# Autodesk Inventor assembly: Assembly
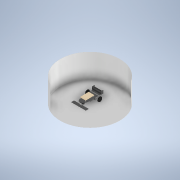
[picture p0: Inventor's stored thumbnail of the model, 180x180]
Saved by Autodesk Inventor 2022 (Build 260153000, 153)
## iProperties
Created: 2021-07-05
Part Number: Assembly
Document SubType Name: Assembly
Designer: ken
Author: ken
## Documents named in this file (12)
- G:\マイドライブ\Projects\lineTracer\inventor\LineTracer.iam
- G:\マイドライブ\Projects\lineTracer\inventor\Tamiya-doubleGearbox.ipt
- G:\マイドライブ\Projects\lineTracer\inventor\Tamiya-SlimTire-36mm.ipt
- G:\マイドライブ\Projects\lineTracer\inventor\Tamiya-ballcaster.ipt
- G:\マイドライブ\Projects\lineTracer\inventor\Akizuki-LineTraceSensor.ipt
- G:\マイドライブ\Projects\lineTracer\inventor\UniversalBoard-72×47.ipt
- G:\マイドライブ\Projects\lineTracer\inventor\spacer-3×10mm.ipt
- G:\マイドライブ\Projects\lineTracer\inventor\spacer-3×20mm.ipt
- G:\マイドライブ\Projects\lineTracer\inventor\18650batteryBox.ipt
- G:\マイドライブ\Projects\lineTracer\inventor\LineTracer-body.ipt
- G:\マイドライブ\Projects\lineTracer\inventor\Tamiya-doubleGearBoxStopper.ipt
- G:\マイドライブ\Projects\lineTracer\inventor\stage.ipt
## Components (17 placed, 11 different names)
1. LineTracer-body:1 — 挿入:22, 挿入:23, 挿入:28, 挿入:29, 挿入:30, 挿入:31, 挿入:34, 挿入:35, 挿入:38, 挿入:39
2. 18650batteryBox:1 — 挿入:34, 挿入:35
3. Tamiya-SlimTire-36mm:1 — 挿入:2
4. Tamiya-SlimTire-36mm:2 — 挿入:1, 正接:2
5. Tamiya-doubleGearbox:1 — 挿入:1, 挿入:2, 挿入:36, 挿入:37
6. Tamiya-doubleGearBoxStopper:1 — 挿入:36, 挿入:37, 挿入:38, 挿入:39
7. UniversalBoard-72×47:1 — 挿入:12, 挿入:13, 挿入:14, 挿入:15
8. Tamiya-ballcaster:1 — 挿入:30, 挿入:31, 正接:3
9. Akizuki-LineTraceSensor:1 — 挿入:19, 挿入:20, 挿入:21
10. spacer-3×10mm:1 — 挿入:12, 挿入:29
11. spacer-3×10mm:2 — 挿入:13
12. spacer-3×10mm:3 — 挿入:15
13. spacer-3×10mm:4 — 挿入:14, 挿入:28
14. spacer-3×20mm:1 — 挿入:21, 挿入:23
15. spacer-3×20mm:2 — 挿入:20
16. spacer-3×20mm:3 — 挿入:19, 挿入:22
17. stage:1 — 正接:2, 正接:3
## Relationships (23: Insert 21, Tangent 2)
- 挿入:1 [Insert]: Tamiya-SlimTire-36mm:2 ↔ Tamiya-doubleGearbox:1
- 挿入:2 [Insert]: Tamiya-SlimTire-36mm:1 ↔ Tamiya-doubleGearbox:1
- 挿入:12 [Insert]: UniversalBoard-72×47:1 ↔ spacer-3×10mm:1
- 挿入:13 [Insert]: UniversalBoard-72×47:1 ↔ spacer-3×10mm:2
- 挿入:14 [Insert]: UniversalBoard-72×47:1 ↔ spacer-3×10mm:4
- 挿入:15 [Insert]: UniversalBoard-72×47:1 ↔ spacer-3×10mm:3
- 挿入:19 [Insert]: Akizuki-LineTraceSensor:1 ↔ spacer-3×20mm:3
- 挿入:20 [Insert]: Akizuki-LineTraceSensor:1 ↔ spacer-3×20mm:2
- 挿入:21 [Insert]: Akizuki-LineTraceSensor:1 ↔ spacer-3×20mm:1
- 挿入:22 [Insert]: LineTracer-body:1 ↔ spacer-3×20mm:3
- 挿入:23 [Insert]: LineTracer-body:1 ↔ spacer-3×20mm:1
- 挿入:28 [Insert]: LineTracer-body:1 ↔ spacer-3×10mm:4
- 挿入:29 [Insert]: LineTracer-body:1 ↔ spacer-3×10mm:1
- 挿入:30 [Insert]: LineTracer-body:1 ↔ Tamiya-ballcaster:1
- 挿入:31 [Insert]: LineTracer-body:1 ↔ Tamiya-ballcaster:1
- 挿入:34 [Insert]: LineTracer-body:1 ↔ 18650batteryBox:1
- 挿入:35 [Insert]: LineTracer-body:1 ↔ 18650batteryBox:1
- 挿入:36 [Insert]: Tamiya-doubleGearbox:1 ↔ Tamiya-doubleGearBoxStopper:1
- 挿入:37 [Insert]: Tamiya-doubleGearbox:1 ↔ Tamiya-doubleGearBoxStopper:1
- 挿入:38 [Insert]: LineTracer-body:1 ↔ Tamiya-doubleGearBoxStopper:1
- 挿入:39 [Insert]: LineTracer-body:1 ↔ Tamiya-doubleGearBoxStopper:1
- 正接:2 [Tangent]: Tamiya-SlimTire-36mm:2 ↔ stage:1
- 正接:3 [Tangent]: Tamiya-ballcaster:1 ↔ stage:1
